# Autodesk Inventor assembly: Hot End Sensors
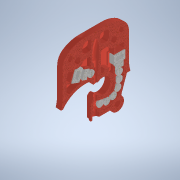
[picture p0: Inventor's stored thumbnail of the model, 180x180]
Saved by Autodesk Inventor 2021 (Build 250183000, 183)
## iProperties
Created: 2021-08-30
Part Number: Hot End Sensors
Document SubType Name: Assembly
Designer: Diego.labarca
Author: Diego.labarca
## Documents named in this file (6)
- E:\Dropbox\Inventor\Impresora 3D\Arreglos Impresora\Mini AB Sensors\Hot End Sensors.iam
- E:\Dropbox\Inventor\Impresora 3D\Arreglos Impresora\Mini AB Sensors\Ball 4mm.ipt
- E:\Dropbox\Inventor\Impresora 3D\Arreglos Impresora\Mini AB Sensors\Mid_Body.ipt
- E:\Dropbox\Inventor\Impresora 3D\Arreglos Impresora\Mini AB Sensors\Iman 5x3.ipt
- E:\Dropbox\Inventor\Impresora 3D\Arreglos Impresora\Mini AB Sensors\Porta Hall Sensor 145-145.ipt
- E:\Dropbox\Inventor\Impresora 3D\Arreglos Impresora\Mini AB Sensors\Hall Sensor.ipt
## Components (13 placed, 5 different names)
1. Mid_Body:1 — Coincidencia:3, Coincidencia:6, Coincidencia:9, Coincidencia:10, Coincidencia:11, Coincidencia:12, Coincidencia:13, Nivelación:3, Nivelación:4, Coincidencia:15, Coincidencia:16
2. Ball 4mm:1 — Coincidencia:2, Nivelación:1, Nivelación:2, Coincidencia:3, Coincidencia:6, Coincidencia:7, Coincidencia:8
3. Ball 4mm:2 — Coincidencia:2, Tangente:2
4. Ball 4mm:3 — Tangente:2, Nivelación:1, Tangente:3
5. Ball 4mm:4 — Nivelación:2, Tangente:3, Tangente:4
6. Ball 4mm:5 — Coincidencia:7, Tangente:4, Tangente:5
7. Ball 4mm:6 — Coincidencia:8, Tangente:5, Tangente:6
8. Iman 5x3:1 — Coincidencia:9, Tangente:6
9. Ball 4mm:7 — Coincidencia:10, Tangente:7
10. Iman 5x3:2 — Coincidencia:11, Tangente:7
11. Porta Hall Sensor 145-145:1 — Coincidencia:12, Coincidencia:13, Nivelación:3
12. Porta Hall Sensor 145-145:2 — Nivelación:4, Coincidencia:15, Coincidencia:16
13. Hall Sensor:1
## Relationships (22: Mate 12, Tangent 6, Flush 4)
- Coincidencia:2 [Mate]: Ball 4mm:1 ↔ Ball 4mm:2
- Tangente:2: Ball 4mm:2 ↔ Ball 4mm:3
- Nivelación:1 [Flush]: Ball 4mm:1 ↔ Ball 4mm:3
- Nivelación:2 [Flush]: Ball 4mm:1 ↔ Ball 4mm:4
- Tangente:3: Ball 4mm:3 ↔ Ball 4mm:4
- Coincidencia:3 [Mate]: Mid_Body:1 ↔ Ball 4mm:1
- Coincidencia:6 [Mate] (2.85 mm): Mid_Body:1 ↔ Ball 4mm:1
- Coincidencia:7 [Mate]: Ball 4mm:1 ↔ Ball 4mm:5
- Tangente:4: Ball 4mm:4 ↔ Ball 4mm:5
- Coincidencia:8 [Mate]: Ball 4mm:1 ↔ Ball 4mm:6
- Tangente:5: Ball 4mm:5 ↔ Ball 4mm:6
- Coincidencia:9 [Mate]: Mid_Body:1 ↔ Iman 5x3:1
- Tangente:6: Ball 4mm:6 ↔ Iman 5x3:1
- Coincidencia:10 [Mate]: Mid_Body:1 ↔ Ball 4mm:7
- Coincidencia:11 [Mate]: Mid_Body:1 ↔ Iman 5x3:2
- Tangente:7: Ball 4mm:7 ↔ Iman 5x3:2
- Coincidencia:12 [Mate]: Mid_Body:1 ↔ Porta Hall Sensor 145-145:1
- Coincidencia:13 [Mate]: Mid_Body:1 ↔ Porta Hall Sensor 145-145:1
- Nivelación:3 [Flush]: Mid_Body:1 ↔ Porta Hall Sensor 145-145:1
- Nivelación:4 [Flush]: Mid_Body:1 ↔ Porta Hall Sensor 145-145:2
- Coincidencia:15 [Mate]: Mid_Body:1 ↔ Porta Hall Sensor 145-145:2
- Coincidencia:16 [Mate]: Mid_Body:1 ↔ Porta Hall Sensor 145-145:2
